# Autodesk Inventor assembly: servo + servo block + 2 in compliant wheel
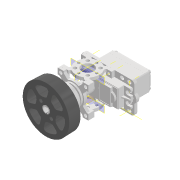
[picture p0: Inventor's stored thumbnail of the model, 180x180]
Saved by Autodesk Inventor 2020 (Build 240168000, 168)
## iProperties
Created: 2020-01-13
Part Number: servo + servo block + 2 in compliant wheel
Document SubType Name: Assembly
Designer: ball
Author: ball
## Documents named in this file (3)
- C:\FTC\FTC8863CAD\2019 Robot\Collection\servo + servo block + 2 in compliant wheel.iam
- C:\FTC\FTC8863CAD\Actobotics\637 parts\637112 servo block 25 spline.iam
- C:\FTC\FTC8863CAD\2019 Robot\Collection\compliant wheel 2 in + 6mm shaft adapterr.iam
## Components (2 placed, 2 different names)
1. 637112 servo block 25 spline:1 [sub-assembly] — Mate:1, Mate:2
2. compliant wheel 2 in + 6mm shaft adapterr:1 [sub-assembly] — Mate:1, Mate:2
## Relationships (2: Mate 2)
- Mate:1: 637112 servo block 25 spline:1 ↔ compliant wheel 2 in + 6mm shaft adapterr:1
- Mate:2: 637112 servo block 25 spline:1 ↔ compliant wheel 2 in + 6mm shaft adapterr:1
